# Autodesk Inventor assembly: HeRoMini2
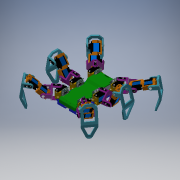
[picture p0: Inventor's stored thumbnail of the model, 180x180]
Saved by Autodesk Inventor 2017 (Build 210142000, 142)
## iProperties
Created: 2018-07-29
Part Number: HeRoMini2
Document SubType Name: Assembly
Designer: Alexander Miller
Author: Alexander Miller
## Documents named in this file (13)
- C:\Users\Alexander Miller\Documents\Git\HeRo-Mini\Hardware\Assembly\HeRoMini2.iam
- C:\Users\Alexander Miller\Documents\Git\HeRo-Mini\Hardware\Part\Design\BODY_BOTTOM.ipt
- C:\Users\Alexander Miller\Documents\Git\HeRo-Mini\Hardware\Assembly\Mainboard.iam
- C:\Users\Alexander Miller\Documents\Git\HeRo-Mini\Hardware\Assembly\LEG.iam
- C:\Users\Alexander Miller\Documents\Git\HeRo-Mini\Hardware\Part\PCB\Regulator1.ipt
- C:\Users\Alexander Miller\Documents\Git\HeRo-Mini\Hardware\Part\PCB\Regulator2.ipt
- C:\Users\Alexander Miller\Documents\Git\HeRo-Mini\Hardware\Assembly\LEG2.iam
- C:\Users\Alexander Miller\Documents\Git\HeRo-Mini\Hardware\Part\PCB\IMU.ipt
- C:\Users\Alexander Miller\Documents\Git\HeRo-Mini\Hardware\Part\Design\BODY_COVER.ipt
- C:\Users\Alexander Miller\Documents\Git\HeRo-Mini\Hardware\Part\Hardware\MAGNET.ipt
- C:\Users\Alexander Miller\Documents\Git\HeRo-Mini\Hardware\Part\Hardware\NUT_2MM.ipt
- C:\Users\Alexander Miller\Documents\Git\HeRo-Mini\Hardware\Part\Hardware\M2_SCREW_10MM.ipt
- C:\Users\Alexander Miller\Documents\Git\HeRo-Mini\Hardware\Part\Hardware\M2_SCREW_6MM.ipt
## Components (53 placed, 12 different names)
1. BODY_BOTTOM:1 — Rigid:1, Rigid:12, Rigid:13, Rigid:14, Rigid:15, Rigid:16, Rigid:21, Rigid:22, Rigid:23, Rigid:24, Rigid:25, Rigid:26, Rigid:27, Rigid:28, Rigid:29, Rigid:30, Rigid:31, Rigid:32, Rigid:33, Rigid:34, Rigid:35, Rigid:36
2. Mainboard:1 [sub-assembly] — Rigid:1, Rigid:2, Rigid:3, Rigid:4, Rigid:5, Rigid:6, Rigid:7, Rigid:8, Rigid:9, Rigid:10, Rigid:11, Rigid:49, Rigid:50, Rigid:51, Rigid:52
3. LEG:1 [sub-assembly] — Rigid:2, Rigid:47, Rigid:48
4. LEG:2 [sub-assembly] — Rigid:3, Rigid:45, Rigid:46
5. LEG:3 [sub-assembly] — Rigid:4, Rigid:37, Rigid:38
6. LEG2:1 [sub-assembly] — Rigid:8, Rigid:43, Rigid:44
7. LEG2:2 [sub-assembly] — Rigid:9, Rigid:39, Rigid:40
8. LEG2:3 [sub-assembly] — Rigid:10, Rigid:41, Rigid:42
9. Regulator1:1 — Rigid:5
10. Regulator1:2 — Rigid:6
11. Regulator2:1 — Rigid:7
12. IMU:1 — Rigid:11
13. BODY_COVER:1 — Rigid:12, Rigid:17, Rigid:18, Rigid:19, Rigid:20
14. MAGNET:1 — Rigid:13
15. MAGNET:2 — Rigid:14
16. MAGNET:3 — Rigid:15
17. MAGNET:4 — Rigid:16
18. MAGNET:5 — Rigid:19
19. MAGNET:6 — Rigid:18
20. MAGNET:7 — Rigid:17
21. MAGNET:8 — Rigid:20
22. NUT_2MM:1 — Rigid:24
23. NUT_2MM:2 — Rigid:22
24. NUT_2MM:3 — Rigid:21
25. NUT_2MM:4 — Rigid:23
26. NUT_2MM:5 — Rigid:36
27. NUT_2MM:6 — Rigid:35
28. NUT_2MM:7 — Rigid:34
29. NUT_2MM:8 — Rigid:33
30. NUT_2MM:9 — Rigid:31
31. NUT_2MM:10 — Rigid:32
32. NUT_2MM:11 — Rigid:29
33. NUT_2MM:12 — Rigid:30
34. NUT_2MM:13 — Rigid:27
35. NUT_2MM:14 — Rigid:28
36. NUT_2MM:15 — Rigid:26
37. NUT_2MM:16 — Rigid:25
38. M2_SCREW_10MM:1 — Rigid:39
39. M2_SCREW_10MM:2 — Rigid:40
40. M2_SCREW_10MM:3 — Rigid:38
41. M2_SCREW_10MM:4 — Rigid:42
42. M2_SCREW_10MM:5 — Rigid:41
43. M2_SCREW_10MM:6 — Rigid:43
44. M2_SCREW_10MM:7 — Rigid:48
45. M2_SCREW_10MM:8 — Rigid:44
46. M2_SCREW_10MM:9 — Rigid:47
47. M2_SCREW_10MM:10 — Rigid:45
48. M2_SCREW_10MM:11 — Rigid:46
49. M2_SCREW_10MM:12 — Rigid:37
50. M2_SCREW_6MM:1 — Rigid:51
51. M2_SCREW_6MM:2 — Rigid:52
52. M2_SCREW_6MM:3 — Rigid:50
53. M2_SCREW_6MM:4 — Rigid:49
## Relationships (52: WeldJoint 52)
- Rigid:1 [WeldJoint]: BODY_BOTTOM:1 ↔ Mainboard:1
- Rigid:2 [WeldJoint] (2.54 mm): Mainboard:1 ↔ LEG:1
- Rigid:3 [WeldJoint] (2.54 mm): Mainboard:1 ↔ LEG:2
- Rigid:4 [WeldJoint] (2.54 mm): Mainboard:1 ↔ LEG:3
- Rigid:5 [WeldJoint]: Mainboard:1 ↔ Regulator1:1
- Rigid:6 [WeldJoint]: Mainboard:1 ↔ Regulator1:2
- Rigid:7 [WeldJoint]: Mainboard:1 ↔ Regulator2:1
- Rigid:8 [WeldJoint] (2.54 mm): Mainboard:1 ↔ LEG2:1
- Rigid:9 [WeldJoint] (2.54 mm): Mainboard:1 ↔ LEG2:2
- Rigid:10 [WeldJoint] (2.54 mm): Mainboard:1 ↔ LEG2:3
- Rigid:11 [WeldJoint]: Mainboard:1 ↔ IMU:1
- Rigid:12 [WeldJoint]: BODY_BOTTOM:1 ↔ BODY_COVER:1
- Rigid:13 [WeldJoint]: BODY_BOTTOM:1 ↔ MAGNET:1
- Rigid:14 [WeldJoint]: BODY_BOTTOM:1 ↔ MAGNET:2
- Rigid:15 [WeldJoint]: BODY_BOTTOM:1 ↔ MAGNET:3
- Rigid:16 [WeldJoint]: BODY_BOTTOM:1 ↔ MAGNET:4
- Rigid:17 [WeldJoint]: BODY_COVER:1 ↔ MAGNET:7
- Rigid:18 [WeldJoint]: BODY_COVER:1 ↔ MAGNET:6
- Rigid:19 [WeldJoint]: BODY_COVER:1 ↔ MAGNET:5
- Rigid:20 [WeldJoint]: BODY_COVER:1 ↔ MAGNET:8
- Rigid:21 [WeldJoint]: BODY_BOTTOM:1 ↔ NUT_2MM:3
- Rigid:22 [WeldJoint]: BODY_BOTTOM:1 ↔ NUT_2MM:2
- Rigid:23 [WeldJoint]: BODY_BOTTOM:1 ↔ NUT_2MM:4
- Rigid:24 [WeldJoint]: BODY_BOTTOM:1 ↔ NUT_2MM:1
- Rigid:25 [WeldJoint]: BODY_BOTTOM:1 ↔ NUT_2MM:16
- Rigid:26 [WeldJoint]: BODY_BOTTOM:1 ↔ NUT_2MM:15
- Rigid:27 [WeldJoint]: BODY_BOTTOM:1 ↔ NUT_2MM:13
- Rigid:28 [WeldJoint]: BODY_BOTTOM:1 ↔ NUT_2MM:14
- Rigid:29 [WeldJoint]: BODY_BOTTOM:1 ↔ NUT_2MM:11
- Rigid:30 [WeldJoint]: BODY_BOTTOM:1 ↔ NUT_2MM:12
- Rigid:31 [WeldJoint]: BODY_BOTTOM:1 ↔ NUT_2MM:9
- Rigid:32 [WeldJoint]: BODY_BOTTOM:1 ↔ NUT_2MM:10
- Rigid:33 [WeldJoint]: BODY_BOTTOM:1 ↔ NUT_2MM:8
- Rigid:34 [WeldJoint]: BODY_BOTTOM:1 ↔ NUT_2MM:7
- Rigid:35 [WeldJoint]: BODY_BOTTOM:1 ↔ NUT_2MM:6
- Rigid:36 [WeldJoint]: BODY_BOTTOM:1 ↔ NUT_2MM:5
- Rigid:37 [WeldJoint]: LEG:3 ↔ M2_SCREW_10MM:12
- Rigid:38 [WeldJoint]: LEG:3 ↔ M2_SCREW_10MM:3
- Rigid:39 [WeldJoint]: LEG2:2 ↔ M2_SCREW_10MM:1
- Rigid:40 [WeldJoint]: LEG2:2 ↔ M2_SCREW_10MM:2
- Rigid:41 [WeldJoint]: LEG2:3 ↔ M2_SCREW_10MM:5
- Rigid:42 [WeldJoint]: LEG2:3 ↔ M2_SCREW_10MM:4
- Rigid:43 [WeldJoint]: LEG2:1 ↔ M2_SCREW_10MM:6
- Rigid:44 [WeldJoint]: LEG2:1 ↔ M2_SCREW_10MM:8
- Rigid:45 [WeldJoint]: LEG:2 ↔ M2_SCREW_10MM:10
- Rigid:46 [WeldJoint]: LEG:2 ↔ M2_SCREW_10MM:11
- Rigid:47 [WeldJoint]: LEG:1 ↔ M2_SCREW_10MM:9
- Rigid:48 [WeldJoint]: LEG:1 ↔ M2_SCREW_10MM:7
- Rigid:49 [WeldJoint]: Mainboard:1 ↔ M2_SCREW_6MM:4
- Rigid:50 [WeldJoint]: Mainboard:1 ↔ M2_SCREW_6MM:3
- Rigid:51 [WeldJoint]: Mainboard:1 ↔ M2_SCREW_6MM:1
- Rigid:52 [WeldJoint]: Mainboard:1 ↔ M2_SCREW_6MM:2
